# Autodesk Inventor assembly: Assembly2
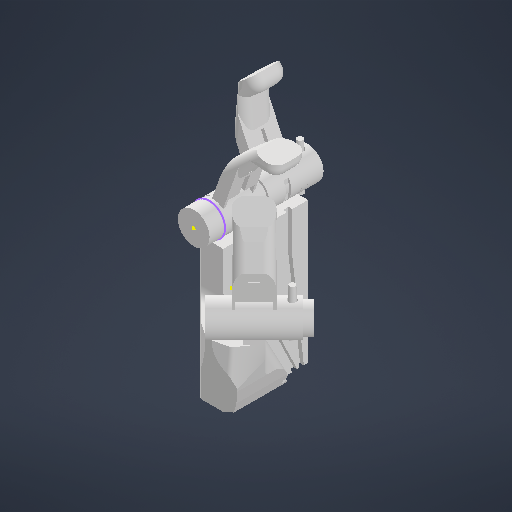
[picture p0: Inventor's stored thumbnail of the model, 512x512]
Saved by Autodesk Inventor 2026.2 (Build 302298010, 298A)
## iProperties
Created: 2026-09-03
Part Number: Assembly2
Document SubType Name: Assembly
Designer: Iulia
Author: Iulia
## Documents named in this file (7)
- C:\Users\Iulia\Desktop\Bio\Assembly2.iam
- C:\Users\Iulia\Desktop\Bio\Bionic Palm.ipt
- C:\Users\Iulia\Desktop\Bio\palm 1 - Copy\2Joint.ipt
- C:\Users\Iulia\Desktop\Bio\palm 1 - Copy\Pin.ipt
- C:\Users\Iulia\Desktop\Bio\palm 1\Pin.ipt
- C:\Users\Iulia\Desktop\Bio\palm 1\Collar.ipt
- C:\Users\Iulia\Desktop\Bio\palm 1\Taper pin.ipt
## Components (10 placed, 5 different names)
1. Bionic Palm:1 — Mate:1, Mate:2, Mate:3, Mate:4, Mate:5, Mate:6, Mate:9
2. 2Joint:1 — Mate:1, Mate:2, Mate:7
3. 2Joint:2 — Mate:3, Mate:4, Mate:13
4. 2Joint:3 — Mate:5, Mate:6, Mate:8, Mate:12
5. Pin:1 — Mate:7, Mate:10
6. Pin:2 — Mate:8, Mate:9, Mate:11
7. Collar:1 — Mate:10, Mate:13, Mate:14
8. Collar:2 — Mate:11, Mate:12, Mate:15
9. Taper pin:1 — Mate:15
10. Taper pin:2 — Mate:14
## Relationships (15: Mate 15)
- Mate:1: Bionic Palm:1 ↔ 2Joint:1
- Mate:2: Bionic Palm:1 ↔ 2Joint:1
- Mate:3: Bionic Palm:1 ↔ 2Joint:2
- Mate:4: Bionic Palm:1 ↔ 2Joint:2
- Mate:5: Bionic Palm:1 ↔ 2Joint:3
- Mate:6: Bionic Palm:1 ↔ 2Joint:3
- Mate:7: 2Joint:1 ↔ Pin:1
- Mate:8: 2Joint:3 ↔ Pin:2
- Mate:9: Bionic Palm:1 ↔ Pin:2
- Mate:10: Pin:1 ↔ Collar:1
- Mate:11: Pin:2 ↔ Collar:2
- Mate:12: 2Joint:3 ↔ Collar:2
- Mate:13: 2Joint:2 ↔ Collar:1
- Mate:14: Collar:1 ↔ Taper pin:2
- Mate:15: Collar:2 ↔ Taper pin:1
